# Autodesk Inventor assembly: s-assy-blacket
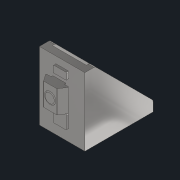
[picture p0: Inventor's stored thumbnail of the model, 180x180]
Saved by Autodesk Inventor 2022 (Build 260153000, 153)
## iProperties
Created: 2021-10-04
Part Number: s-assy-blacket
Document SubType Name: Assembly
Designer: Yuta Kage
Author: Yuta Kage
## Documents named in this file (4)
- C:\Users\yuta0\Downloads\0928\s-assy-blacket.iam
- C:\Users\yuta0\Downloads\0928\HBLFSN5h5.ipt
- C:\Users\yuta0\Downloads\0928\HNTT5-5.ipt
- C:\Users\yuta0\Desktop\lab\Nicebot5 Drawing to Ogura\NIcebot5_J1-J3\CB5_10.ipt
## Components (5 placed, 3 different names)
1. HBLFSN5h5:1 — メイト:1, メイト:2, メイト:3, メイト:4, 角度:1, 角度:2, メイト:5, メイト:6, メイト:7, メイト:8
2. HNTT5-5:1 — メイト:1, メイト:2, 角度:2
3. HNTT5-5:2 — メイト:3, メイト:4, 角度:1
4. CB5_10:1 — メイト:5, メイト:6
5. CB5_10:2 — メイト:7, メイト:8
## Relationships (10: Mate 8, Angle 2)
- メイト:1 [Mate]: HBLFSN5h5:1 ↔ HNTT5-5:1
- メイト:2 [Mate] (2 mm): HBLFSN5h5:1 ↔ HNTT5-5:1
- メイト:3 [Mate]: HBLFSN5h5:1 ↔ HNTT5-5:2
- メイト:4 [Mate] (2 mm): HBLFSN5h5:1 ↔ HNTT5-5:2
- 角度:1 [Angle] (0 deg): HBLFSN5h5:1 ↔ HNTT5-5:2
- 角度:2 [Angle] (0 deg): HBLFSN5h5:1 ↔ HNTT5-5:1
- メイト:5 [Mate]: HBLFSN5h5:1 ↔ CB5_10:1
- メイト:6 [Mate]: HBLFSN5h5:1 ↔ CB5_10:1
- メイト:7 [Mate]: HBLFSN5h5:1 ↔ CB5_10:2
- メイト:8 [Mate]: HBLFSN5h5:1 ↔ CB5_10:2
